# Autodesk Inventor assembly: frEonV2
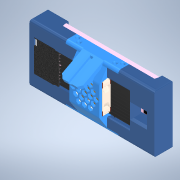
[picture p0: Inventor's stored thumbnail of the model, 180x180]
Saved by Autodesk Inventor 2020 (Build 240168000, 168)
## iProperties
Created: 2021-04-14
Part Number: frEonV2
Document SubType Name: Assembly
Designer: dkiiv
Author: dkiiv
## Documents named in this file (10)
- D:\CAD\leeco-freon\V2\frEonV2.iam
- D:\CAD\leeco-freon\V2\eonPCB.ipt
- D:\CAD\leeco-freon\V2\heatsink.ipt
- D:\CAD\leeco-freon\V2\leeco.ipt
- D:\CAD\leeco-freon\V2\noctua fan\NF-A4x10_Noctua_40mm.iam
- D:\CAD\leeco-freon\V2\printed parts\left.ipt
- D:\CAD\leeco-freon\V2\printed parts\right.ipt
- D:\CAD\leeco-freon\V2\printed parts\middle\IR\middle28DEG-IR.ipt
- D:\CAD\leeco-freon\V2\printed parts\middle\IR-less\middle28DEG.ipt
- D:\CAD\leeco-freon\V2\printed parts\eonPCBcover.ipt
## Components (9 placed, 9 different names)
1. eonPCB:1 — Mate:3, Mate:4, Mate:5, Mate:11
2. heatsink:1 — Mate:1, Flush:1, Flush:2, Flush:3, Mate:15
3. leeco:1 — Mate:1, Flush:1, Flush:3, Mate:3, Mate:4, Mate:5, Mate:6, Mate:7, Mate:8, Mate:10
4. NF-A4x10_Noctua_40mm:1 [sub-assembly] — Flush:2, Mate:15, Flush:7
5. left:1 — Mate:6, Mate:7, Flush:5, Mate:10, Flush:6, Flush:8
6. right:1 — Mate:8, Flush:5, Mate:11, Mate:13, Mate:14, Flush:9, Mate:16, Flush:10, Mate:17, Mate:18
7. middle28DEG-IR:1 — Flush:6, Mate:13, Mate:14, Flush:7
8. middle28DEG:1 — Flush:8, Flush:9, Mate:16
9. eonPCBcover:1 — Flush:10, Mate:17, Mate:18
## Relationships (24: Mate 15, Flush 9)
- Mate:1: heatsink:1 ↔ leeco:1
- Flush:1 (7 mm): heatsink:1 ↔ leeco:1
- Flush:2 (10 mm): heatsink:1 ↔ NF-A4x10_Noctua_40mm:1
- Flush:3 (20 mm): heatsink:1 ↔ leeco:1
- Mate:3: eonPCB:1 ↔ leeco:1
- Mate:4: eonPCB:1 ↔ leeco:1
- Mate:5: eonPCB:1 ↔ leeco:1
- Mate:6: leeco:1 ↔ left:1
- Mate:7: leeco:1 ↔ left:1
- Mate:8: leeco:1 ↔ right:1
- Flush:5: left:1 ↔ right:1
- Mate:10: leeco:1 ↔ left:1
- Mate:11 (3.4 mm): eonPCB:1 ↔ right:1
- Flush:6: left:1 ↔ middle28DEG-IR:1
- Mate:13: right:1 ↔ middle28DEG-IR:1
- Mate:14: right:1 ↔ middle28DEG-IR:1
- Mate:15: heatsink:1 ↔ NF-A4x10_Noctua_40mm:1
- Flush:7: NF-A4x10_Noctua_40mm:1 ↔ middle28DEG-IR:1
- Flush:8: left:1 ↔ middle28DEG:1
- Flush:9: right:1 ↔ middle28DEG:1
- Mate:16: right:1 ↔ middle28DEG:1
- Flush:10: right:1 ↔ eonPCBcover:1
- Mate:17: right:1 ↔ eonPCBcover:1
- Mate:18: right:1 ↔ eonPCBcover:1
